# Autodesk Inventor assembly: confirmat
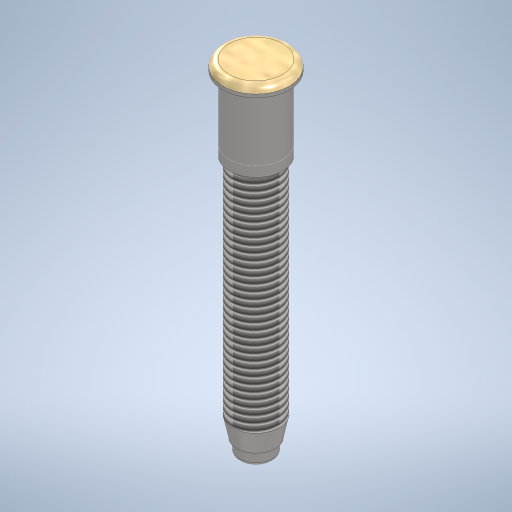
[picture p0: Inventor's stored thumbnail of the model, 512x512]
Saved by Autodesk Inventor 2024 (Build 280153000, 153)
## iProperties
Created: 2021-09-13
Part Number: confirmat
Document SubType Name: Assembly
Designer: RokasM
Author: RokasM
## iProperties of the stored document MemberDocs/xImj0hbweFkl04es5Hnkdc30dCd
Created: 2021-09-13
Document SubType Name: Assembly
Designer: RokasM
Author: RokasM
## iProperties of the stored document MemberDocs/x1ds3cb3fJ0ym1xpzAsnnndfs4d
Created: 2021-09-13
Document SubType Name: Assembly
Designer: RokasM
Author: RokasM
## iProperties of the stored document MemberDocs/x010x0nd3Lku2kwdpYconikasCg
Created: 2021-09-13
Document SubType Name: Assembly
Designer: RokasM
Author: RokasM
## iProperties of the stored document MemberDocs/xAiupnz12G0phwnfj5vlhhd2xTg
Created: 2021-09-13
Document SubType Name: Assembly
Designer: RokasM
Author: RokasM
## iProperties of the stored document MemberDocs/xMctp34eyP0wv4mvp3mfvbqbjQb
Created: 2021-09-13
Document SubType Name: Assembly
Designer: RokasM
Author: RokasM
## iProperties of the stored document MemberDocs/xJ5liesjfE0fezg1iMxix3unaJh
Created: 2021-09-13
Document SubType Name: Assembly
Designer: RokasM
Author: RokasM
## iProperties of the stored document MemberDocs/xIq4e4guvM0zhrskdWfl5medjXf
Created: 2021-09-13
Document SubType Name: Assembly
Designer: RokasM
Author: RokasM
## iProperties of the stored document MemberDocs/xLq2ltr5xMkvcgtdcYfkbyx1jAf
Created: 2021-09-13
Document SubType Name: Assembly
Designer: RokasM
Author: RokasM
## iProperties of the stored document MemberDocs/xRfpjvr2zBs5pka2iMdk3sdtj2c
Created: 2021-09-13
Document SubType Name: Assembly
Designer: RokasM
Author: RokasM
## iProperties of the stored document MemberDocs/xOjh25vdmLkmnttkc4mjnwtcp1e
Created: 2021-09-13
Document SubType Name: Assembly
Designer: RokasM
Author: RokasM
## iProperties of the stored document MemberDocs/xUduqqpceDck433wmXpot2keqPb
Created: 2021-09-13
Document SubType Name: Assembly
Designer: RokasM
Author: RokasM
## iProperties of the stored document MemberDocs/xRlyfi5lcGkwpprdkZybrvssk3e
Created: 2021-09-13
Document SubType Name: Assembly
Designer: RokasM
Author: RokasM
## iProperties of the stored document MemberDocs/xWxnbla3rKkhdlsyh2gk5joh2Bg
Created: 2021-09-13
Document SubType Name: Assembly
Designer: RokasM
Author: RokasM
## iProperties of the stored document MemberDocs/xYk5fxr2kFsnyr2xuUsetzmlgUb
Created: 2021-09-13
Document SubType Name: Assembly
Designer: RokasM
Author: RokasM
## Documents named in this file (7)
- C:\W4INV 2024 Design\LIBRARY\Fixed joints\Confirmat\Confirmat\confirmat.iam
- C:\W4INV 2024 Design\LIBRARY\Fixed joints\Confirmat\Confirmat\confirmat.ipt
- C:\W4INV 2024 Design\LIBRARY\Fixed joints\Confirmat\Confirmat\Cap.ipt
- C:\W4INV 2022 Design\LIBRARY\NEW\Fixed joints\Confirmat\confirmat.ipt
- C:\W4INV 2022 Design\LIBRARY\NEW\Fixed joints\Confirmat\Cap.ipt
- C:\W4INV 2022 Design\LIBRARY\Fixed joints\Confirmat\Confirmat\confirmat.ipt
- C:\W4INV 2022 Design\LIBRARY\Fixed joints\Confirmat\Confirmat\Cap.ipt
## Components (2 placed, 2 different names)
1. confirmat:1
2. Cap:1 — Flush:1
## Relationships (1: Flush 1)
- Flush:1: Cap:1
## Named parameters: Pillar_Board_Thickness = 12 mm
